# Autodesk Inventor assembly: Main assembly
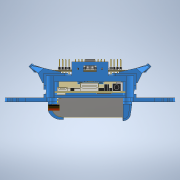
[picture p0: Inventor's stored thumbnail of the model, 180x180]
Saved by Autodesk Inventor 2022 (Build 260153000, 153)
## iProperties
Created: 2023-01-31
Part Number: Main assembly
Document SubType Name: Assembly
Designer: scott
Author: scott
## Documents named in this file (11)
- C:\Users\scott\OneDrive\Documents\Cat project\Git_repository\Flinders_OpenCat\CAD components\Main assembly.iam
- C:\Users\scott\OneDrive\Documents\Cat project\Git_repository\Flinders_OpenCat\CAD components\Pi_mount.ipt
- C:\Users\scott\OneDrive\Documents\Cat project\Git_repository\Flinders_OpenCat\CAD components\Pi_lid.ipt
- C:\Users\scott\OneDrive\Documents\Cat project\Git_repository\Flinders_OpenCat\CAD components\Raspberry PI 3 Model A+ - Simple.ipt
- C:\Users\scott\OneDrive\Documents\Cat project\Git_repository\Flinders_OpenCat\CAD components\Base_modded.ipt
- C:\Users\scott\OneDrive\Documents\Cat project\Git_repository\Flinders_OpenCat\CAD components\Battery_temp.ipt
- C:\Users\scott\OneDrive\Documents\Cat project\Git_repository\Flinders_OpenCat\CAD components\Battery mount front.ipt
- C:\Users\scott\OneDrive\Documents\Cat project\Git_repository\Flinders_OpenCat\CAD components\battery mount rear.ipt
- C:\Users\scott\OneDrive\Documents\Cat project\Git_repository\Flinders_OpenCat\CAD components\MPU_6050.ipt
- C:\Users\scott\OneDrive\Documents\Cat project\Git_repository\Flinders_OpenCat\CAD components\815 Servo Driver 16 Channel.ipt
- C:\Users\scott\OneDrive\Documents\Cat project\Git_repository\Flinders_OpenCat\CAD components\Braces.ipt
## Components (12 placed, 10 different names)
1. Pi_mount:1 — Mate:1, Mate:2, Mate:3, Mate:4, Mate:6, Mate:7, Mate:8, Mate:9, Mate:10, Mate:11, Mate:12, Mate:13
2. Pi_lid:1 — Mate:1, Mate:2, Mate:5, Mate:20, Mate:21, Mate:22, Mate:23, Mate:24, Mate:25, Mate:26, Mate:27, Mate:28, Mate:29
3. Raspberry PI 3 Model A+ - Simple:1 — Mate:3, Mate:4, Mate:5, Mate:6
4. Base_modded:1 — Mate:7, Mate:8, Mate:9, Mate:14, Mate:15, Mate:17
5. Base_modded:2 — Mate:10, Mate:11, Mate:12, Mate:18, Mate:19
6. Battery_temp:1 — Mate:13, Flush:1, Mate:16
7. Battery mount front:1 — Mate:14, Mate:15, Flush:1, Mate:16, Mate:17
8. battery mount rear:1 — Mate:18, Mate:19
9. MPU_6050:1 — Mate:20, Mate:21, Mate:22
10. 815 Servo Driver 16 Channel:1 — Mate:23, Mate:24, Mate:25
11. Braces:1 — Mate:28, Mate:29
12. Braces:3 — Mate:26, Mate:27
## Relationships (30: Mate 29, Flush 1)
- Mate:1: Pi_mount:1 ↔ Pi_lid:1
- Mate:2: Pi_mount:1 ↔ Pi_lid:1
- Mate:3: Pi_mount:1 ↔ Raspberry PI 3 Model A+ - Simple:1
- Mate:4: Pi_mount:1 ↔ Raspberry PI 3 Model A+ - Simple:1
- Mate:5: Pi_lid:1 ↔ Raspberry PI 3 Model A+ - Simple:1
- Mate:6: Pi_mount:1 ↔ Raspberry PI 3 Model A+ - Simple:1
- Mate:7: Pi_mount:1 ↔ Base_modded:1
- Mate:8: Pi_mount:1 ↔ Base_modded:1
- Mate:9: Pi_mount:1 ↔ Base_modded:1
- Mate:10: Pi_mount:1 ↔ Base_modded:2
- Mate:11: Pi_mount:1 ↔ Base_modded:2
- Mate:12: Pi_mount:1 ↔ Base_modded:2
- Mate:13: Pi_mount:1 ↔ Battery_temp:1
- Mate:14: Base_modded:1 ↔ Battery mount front:1
- Mate:15: Base_modded:1 ↔ Battery mount front:1
- Flush:1: Battery_temp:1 ↔ Battery mount front:1
- Mate:16: Battery_temp:1 ↔ Battery mount front:1
- Mate:17: Base_modded:1 ↔ Battery mount front:1
- Mate:18: Base_modded:2 ↔ battery mount rear:1
- Mate:19: Base_modded:2 ↔ battery mount rear:1
- Mate:20: Pi_lid:1 ↔ MPU_6050:1
- Mate:21: Pi_lid:1 ↔ MPU_6050:1
- Mate:22: Pi_lid:1 ↔ MPU_6050:1
- Mate:23: Pi_lid:1 ↔ 815 Servo Driver 16 Channel:1
- Mate:24: Pi_lid:1 ↔ 815 Servo Driver 16 Channel:1
- Mate:25: Pi_lid:1 ↔ 815 Servo Driver 16 Channel:1
- Mate:26: Pi_lid:1 ↔ Braces:3
- Mate:27: Pi_lid:1 ↔ Braces:3
- Mate:28: Pi_lid:1 ↔ Braces:1
- Mate:29: Pi_lid:1 ↔ Braces:1
